# Autodesk Inventor assembly: Trim Pot Assembly
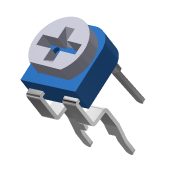
[picture p0: Inventor's stored thumbnail of the model, 180x180]
Saved by Autodesk Inventor 2014 (Build 180170000, 170)
## iProperties
Created: 2015-10-12
Part Number: Trim Pot Assembly
Document SubType Name: Assembly
Designer: Tom
Author: Tom
## Documents named in this file (6)
- C:\Users\tom\Documents\Inventor\Component Library\Trim Pot\Trim Pot Assembly.iam
- C:\Users\tom\Documents\Inventor\Control Glove\trim pot_ body.ipt
- C:\Users\tom\Documents\Inventor\Control Glove\wiper.ipt
- C:\Users\tom\Documents\Inventor\Control Glove\pin_1.ipt
- C:\Users\tom\Documents\Inventor\Control Glove\pin_1_2.ipt
- C:\Users\tom\Documents\Inventor\Control Glove\pin_2.ipt
## Components (5 placed, 5 different names)
1. trim pot_ body:1 — Rotational:1, Flush:1, Flush:4, Mate:1, Mate:2, Mate:3, Mate:4, Mate:5
2. wiper:1 — Rotational:1
3. pin_1:1 — Flush:1, Flush:4, Mate:1, Flush:6, Flush:7
4. pin_1_2:1 — Mate:5, Flush:6, Flush:7
5. pin_2:1 — Mate:2, Mate:3, Mate:4
## Relationships (11: Flush 5, Mate 5, RevoluteJoint 1)
- Rotational:1 [RevoluteJoint]: trim pot_ body:1 ↔ wiper:1
- Flush:1 (1.143 mm): trim pot_ body:1 ↔ pin_1:1
- Flush:4 (0.381 mm): trim pot_ body:1 ↔ pin_1:1
- Mate:1 (0.254 mm): trim pot_ body:1 ↔ pin_1:1
- Flush:5 (-19.4564 mm)
- Mate:2 (0.127 mm): trim pot_ body:1 ↔ pin_2:1
- Mate:3: trim pot_ body:1 ↔ pin_2:1
- Mate:4: trim pot_ body:1 ↔ pin_2:1
- Mate:5: trim pot_ body:1 ↔ pin_1_2:1
- Flush:6 (-5.08 mm): pin_1:1 ↔ pin_1_2:1
- Flush:7: pin_1:1 ↔ pin_1_2:1
